# Autodesk Inventor assembly: Montagem_sistema_simplificado
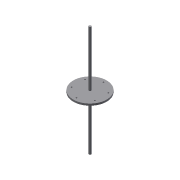
[picture p0: Inventor's stored thumbnail of the model, 180x180]
Saved by Autodesk Inventor 2018 (Build 220112000, 112)
## iProperties
Created: 2019-05-25
Part Number: Montagem_sistema_simplificado
Material: Genérico
Document SubType Name: Assembly
Designer: vinig
Author: vinig
## Documents named in this file (3)
- C:\Users\vinig\OneDrive\Ambiente de Trabalho\Vinícius\TCC\Computacional\Desenho_CAD\Montagem_sistema_simplificado.iam
- C:\Users\vinig\OneDrive\Ambiente de Trabalho\Vinícius\TCC\Computacional\Desenho_CAD\Disco.ipt
- C:\Users\vinig\OneDrive\Ambiente de Trabalho\Vinícius\TCC\Computacional\Desenho_CAD\Eixo_simplificado.ipt
## Components (2 placed, 2 different names)
1. Disco:1 — Rotativa:1
2. Eixo_simplificado:1 — Rotativa:1
## Relationships (1: RevoluteJoint 1)
- Rotativa:1 [RevoluteJoint]: Disco:1 ↔ Eixo_simplificado:1
